# Autodesk Inventor assembly: fms 90mm edf
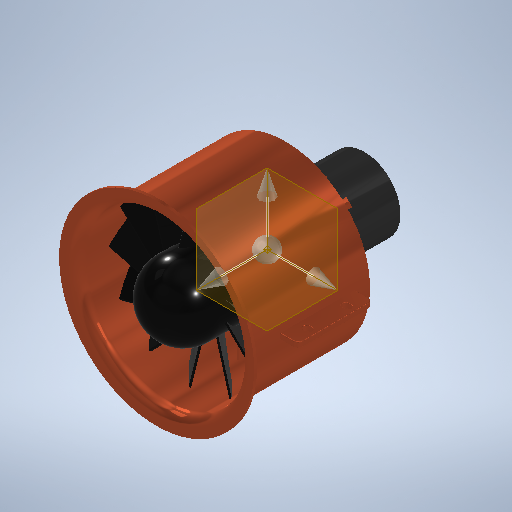
[picture p0: Inventor's stored thumbnail of the model, 512x512]
Saved by Autodesk Inventor 2026.2 (Build 302298010, 298A)
## iProperties
Created: 2026-03-12
Part Number: fms 90mm edf
Document SubType Name: Assembly
Designer: tngzj
Mass: 550 g
Surface Area: 1008.7 cm^2
Volume: 196.46 cm^3
Author: tngzj
## Documents named in this file (4)
- C:\Transformer-rl-retro-propulsion\CAD\EDF Drone v1\Fan\fms 90mm edf.iam
- C:\Transformer-rl-retro-propulsion\CAD\EDF Drone v1\Fan\EDF Fan Can.ipt
- C:\Transformer-rl-retro-propulsion\CAD\EDF Drone v1\Fan\EDF Fan.ipt
- C:\Transformer-rl-retro-propulsion\CAD\EDF Drone v1\Fan\EDF Motor 4068.ipt
## Components (3 placed, 3 different names)
1. EDF Fan Can:1 — Mate:1, Flush:1
2. EDF Fan:1 — Mate:2, Mate:3
3. EDF Motor 4068:1 — Mate:1, Flush:1, Mate:2, Mate:3
## Relationships (4: Mate 3, Flush 1)
- Mate:1: EDF Fan Can:1 ↔ EDF Motor 4068:1
- Flush:1 (-5 mm): EDF Fan Can:1 ↔ EDF Motor 4068:1
- Mate:2: EDF Fan:1 ↔ EDF Motor 4068:1
- Mate:3: EDF Fan:1 ↔ EDF Motor 4068:1
